# Autodesk Inventor assembly: Vex Traction Wheel 8x2
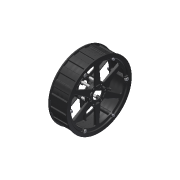
[picture p0: Inventor's stored thumbnail of the model, 180x180]
Saved by Autodesk Inventor 2013 (Build 170138000, 138)
## iProperties
Created: 2012-12-09
Part Number: Vex Traction Wheel 8x2
Document SubType Name: Assembly
Designer: Nemo
Mass: 482.386 g
Surface Area: 1934.24 cm^2
Volume: 408.501 cm^3
Density: 1.18087 g/cm^3
Author: Nemo
## Documents named in this file (6)
- H:\Nemo\Documents\Robotics\COTS Parts\Wheels\VexPro Traction Wheels\Vex Traction Wheel 8x2.iam
- H:\Nemo\Documents\Robotics\COTS Parts\Wheels\VexPro Traction Wheels\Components\Traction Wheel Body 8in.ipt
- H:\Nemo\Documents\Robotics\COTS Parts\Fasteners\8-32 locknut.ipt
- H:\Nemo\Documents\Robotics\COTS Parts\Wheels\VexPro Traction Wheels\Components\Traction Wheel extension 8in.ipt
- H:\Nemo\Documents\Robotics\COTS Parts\Fasteners\Hex Standoff 8-32 x1750.ipt
- H:\Nemo\Documents\Robotics\COTS Parts\Fasteners\8-32 SHCS x2250.ipt
## Components (22 placed, 5 different names)
1. Traction Wheel Body 8in:1 — Mate:1, Mate:2, Angle:1, Insert:1, Mate:4, Insert:5, Angle:2, Mate:6, Mate:7, Insert:6
2. Traction Wheel Body 8in:2 — Mate:3, Mate:4, Insert:4, Angle:3, Mate:11, Insert:7
3. Traction Wheel extension 8in:1 — Mate:5, Mate:6, Mate:7, Flush:1, Mate:9, Mate:10
4. Traction Wheel extension 8in:2 — Mate:8, Mate:9, Mate:10, Mate:11
5. Hex Standoff 8-32 x1750:1 — Angle:1, Insert:1
6. Hex Standoff 8-32 x1750:2
7. Hex Standoff 8-32 x1750:3
8. Hex Standoff 8-32 x1750:4
9. Hex Standoff 8-32 x1750:5
10. Hex Standoff 8-32 x1750:6
11. 8-32 SHCS x2250:1 — Insert:7
12. 8-32 SHCS x2250:2 — Insert:6
13. 8-32 locknut:2 — Insert:4, Angle:3
14. 8-32 locknut:1 — Insert:5, Angle:2
15. 8-32 SHCS x2250:3
16. 8-32 SHCS x2250:4
17. 8-32 locknut:3
18. 8-32 locknut:4
19. 8-32 SHCS x2250:5
20. 8-32 SHCS x2250:6
21. 8-32 locknut:5
22. 8-32 locknut:6
## Component patterns: (6 elements, first: Hex Standoff 8-32 x1750:1), (3 elements, first: 8-32 SHCS x2250:1 + 8-32 SHCS x2250:2 + 8-32 locknut:2 + 8-32 locknut:1)
## Relationships (20: Mate 11, Insert 5, Angle 3, Flush 1)
- Mate:1: Traction Wheel Body 8in:1
- Mate:2: Traction Wheel Body 8in:1
- Angle:1 (0 deg): Traction Wheel Body 8in:1 ↔ Hex Standoff 8-32 x1750:1
- Insert:1: Traction Wheel Body 8in:1 ↔ Hex Standoff 8-32 x1750:1
- Mate:3: Traction Wheel Body 8in:2
- Mate:4: Traction Wheel Body 8in:1 ↔ Traction Wheel Body 8in:2
- Insert:4: Traction Wheel Body 8in:2 ↔ 8-32 locknut:2
- Insert:5: Traction Wheel Body 8in:1 ↔ 8-32 locknut:1
- Angle:2 (0 deg): Traction Wheel Body 8in:1 ↔ 8-32 locknut:1
- Angle:3 (0 deg): Traction Wheel Body 8in:2 ↔ 8-32 locknut:2
- Mate:5: Traction Wheel extension 8in:1
- Mate:6: Traction Wheel Body 8in:1 ↔ Traction Wheel extension 8in:1
- Mate:7: Traction Wheel Body 8in:1 ↔ Traction Wheel extension 8in:1
- Flush:1: Traction Wheel extension 8in:1
- Mate:8: Traction Wheel extension 8in:2
- Mate:9: Traction Wheel extension 8in:1 ↔ Traction Wheel extension 8in:2
- Mate:10: Traction Wheel extension 8in:1 ↔ Traction Wheel extension 8in:2
- Mate:11: Traction Wheel Body 8in:2 ↔ Traction Wheel extension 8in:2
- Insert:6: Traction Wheel Body 8in:1 ↔ 8-32 SHCS x2250:2
- Insert:7: Traction Wheel Body 8in:2 ↔ 8-32 SHCS x2250:1
